# Autodesk Inventor assembly: Final assembly of buggy bot
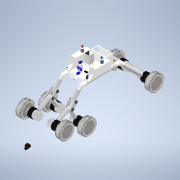
[picture p0: Inventor's stored thumbnail of the model, 180x180]
Saved by Autodesk Inventor 2021 (Build 250183000, 183)
## iProperties
Created: 2021-07-16
Part Number: Final assembly of buggy bot
Document SubType Name: Assembly
Designer: HP
Mass: 47107.8 g
Surface Area: 24762.8 cm^2
Volume: 9232.38 cm^3
Density: 5.10246 g/cm^3
Author: HP
## Documents named in this file (26)
- F:\autodesk inventor\MII\Final assembly of buggy bot.iam
- F:\autodesk inventor\MII\Body.ipt
- F:\autodesk inventor\MII\pvc up.ipt
- F:\autodesk inventor\MII\45elbowfinal.ipt
- F:\autodesk inventor\MII\PVC front 1.ipt
- F:\autodesk inventor\MII\HOLDERPVC.ipt
- F:\autodesk inventor\MII\Dc catcher.ipt
- F:\autodesk inventor\MII\DC.ipt
- F:\autodesk inventor\MII\wheel.ipt
- F:\autodesk inventor\MII\Servo.ipt
- F:\autodesk inventor\MII\smoke.ipt
- F:\autodesk inventor\MII\tilt.ipt
- F:\autodesk inventor\MII\dc to dc.ipt
- F:\autodesk inventor\MII\hbridge.ipt
- F:\autodesk inventor\MII\holder.ipt
- F:\autodesk inventor\MII\bolt.ipt
- F:\autodesk inventor\MII\elbow.ipt
- F:\autodesk inventor\MII\PVC front.ipt
- F:\autodesk inventor\Buggy bot assembly file\Arduino board.ipt
- F:\autodesk inventor\MII\ultrasonic sensor.ipt
- F:\autodesk inventor\MII\temperature sensor.ipt
- F:\autodesk inventor\Water tank.ipt
- F:\autodesk inventor\MII\LED - Copy.ipt
- F:\autodesk inventor\MII\Buzzer.ipt
- F:\autodesk inventor\MII\LED.ipt
- F:\autodesk inventor\Obstacle stone.ipt
## Components (57 placed, 25 different names)
1. Body:1 — Tangent:1, Tangent:2, Flush:1, Flush:2, Angle:2, Tangent:6, Tangent:7, Flush:3, Angle:6, Mate:88, Mate:89, Rigid:8, Angle:7, Angle:10, Angle:11, Insert:1, Rigid:17, Mate:157, Rigid:19, Rotational:2, Rigid:20, Rigid:21, Rigid:22, Rigid:23, Rotational:3
2. pvc up:1 — Tangent:1, Tangent:2, Flush:1, Flush:2, Mate:1, Mate:2, Mate:3, Mate:4
3. 45elbowfinal:1 — Mate:3, Mate:4, Mate:10, Mate:11
4. 45elbowfinal:2 — Mate:1, Mate:2, Mate:13, Mate:14
5. PVC front 1:2 — Mate:10, Mate:11, Mate:43, Rigid:6
6. HOLDERPVC:1 — Mate:13, Mate:14, Mate:92, Mate:93, Tangent:8
7. Dc catcher:2 — Mate:43, Rigid:6, Angle:2, Mate:47, Mate:48
8. DC:5 — Mate:47, Mate:48, Mate:49, Mate:50
9. wheel:1 — Mate:49, Mate:50, Angle:12, Angle:13
10. pvc up:2 — Tangent:6, Tangent:7, Flush:3, Mate:69, Mate:70, Mate:78, Mate:79
11. 45elbowfinal:3 — Mate:69, Mate:70, Mate:71, Mate:72
12. PVC front 1:3 — Mate:71, Mate:72, Mate:73, Rigid:7
13. Dc catcher:9 — Mate:73, Rigid:7, Angle:6, Mate:74, Mate:75
14. DC:8 — Mate:74, Mate:75, Mate:76, Mate:77
15. wheel:6 — Mate:76, Mate:77, Angle:15
16. 45elbowfinal:4 — Mate:78, Mate:79, Mate:80, Mate:81
17. HOLDERPVC:2 — Mate:80, Mate:81, Mate:109, Mate:110, Tangent:11, Tangent:12, Mate:111
18. Servo:1 — Rigid:22
19. smoke:1 — Mate:88, Insert:1
20. tilt:1 — Mate:89
21. dc to dc:1 — Rigid:8
22. hbridge:1 — Mate:157
23. holder:1 — Mate:92, Mate:94, Mate:95, Angle:7, Angle:8, Tangent:8, Mate:97, Mate:100, Tangent:9
24. holder:2 — Mate:93, Mate:96, Angle:8, Mate:98, Tangent:10
25. holder:3 — Mate:110, Tangent:11, Angle:10, Mate:112, Mate:113, Mate:115, Mate:116
26. holder:4 — Mate:109, Tangent:12, Angle:11, Mate:114, Tangent:13
27. bolt:1 — Mate:94, Mate:95, Mate:96
28. elbow:1 — Mate:113, Mate:114, Tangent:13, Mate:128, Mate:129, Mate:131, Mate:132
29. elbow:2 — Mate:97, Mate:98, Mate:99, Tangent:9, Tangent:10, Mate:125, Mate:126, Mate:130, Mate:133
30. bolt:2 — Mate:99, Mate:100
31. bolt:3 — Mate:111, Mate:112
32. bolt:4 — Mate:115, Mate:116
33. PVC front:1 — Mate:125, Mate:126, Mate:127, Mate:146
34. Dc catcher:10 — Mate:127, Mate:146
35. DC:9
36. wheel:7 — Angle:12, Angle:13, Angle:14
37. PVC front:4 — Mate:128, Mate:131, Mate:142, Mate:145
38. PVC front:5 — Mate:130, Mate:133, Mate:140, Mate:141
39. PVC front:6 — Mate:129, Mate:132, Mate:143, Mate:144
40. Dc catcher:11 — Mate:140, Mate:141
41. DC:10 — Mate:147, Mate:148
42. Dc catcher:12 — Mate:143, Mate:144
43. DC:11 — Mate:149, Mate:151
44. Dc catcher:13 — Mate:142, Mate:145
45. DC:12 — Mate:150, Mate:152
46. wheel:8 — Angle:14, Mate:147, Mate:148
47. wheel:9 — Mate:150, Mate:152, Angle:15, Angle:16
48. wheel:10 — Mate:149, Mate:151, Angle:16
49. Arduino board:1 — Rigid:17
50. ultrasonic sensor:1 — Insert:2
51. temperature sensor:1 — Rigid:20
52. Water tank:1 — Rigid:19
53. LED - Copy:1 — Rotational:2
54. Buzzer:1 — Rigid:21
55. Servo:2 — Rigid:23, Insert:2
56. LED:1 — Rotational:3
57. Obstacle stone:1
## Relationships (118: Mate 78, WeldJoint 12, Angle 11, Tangent 10, Flush 3, Insert 2, RevoluteJoint 2)
- Tangent:1: Body:1 ↔ pvc up:1
- Tangent:2: Body:1 ↔ pvc up:1
- Flush:1: Body:1 ↔ pvc up:1
- Flush:2: Body:1 ↔ pvc up:1
- Mate:1: pvc up:1 ↔ 45elbowfinal:2
- Mate:2: pvc up:1 ↔ 45elbowfinal:2
- Mate:3: pvc up:1 ↔ 45elbowfinal:1
- Mate:4: pvc up:1 ↔ 45elbowfinal:1
- Mate:10: 45elbowfinal:1 ↔ PVC front 1:2
- Mate:11: 45elbowfinal:1 ↔ PVC front 1:2
- Mate:13: 45elbowfinal:2 ↔ HOLDERPVC:1
- Mate:14: 45elbowfinal:2 ↔ HOLDERPVC:1
- Mate:43: PVC front 1:2 ↔ Dc catcher:2
- Rigid:6 [WeldJoint]: PVC front 1:2 ↔ Dc catcher:2
- Angle:2 (0 deg): Body:1 ↔ Dc catcher:2
- Mate:47: Dc catcher:2 ↔ DC:5
- Mate:48: Dc catcher:2 ↔ DC:5
- Mate:49: DC:5 ↔ wheel:1
- Mate:50 (5 mm): DC:5 ↔ wheel:1
- Tangent:6: Body:1 ↔ pvc up:2
- Tangent:7: Body:1 ↔ pvc up:2
- Flush:3: Body:1 ↔ pvc up:2
- Mate:69: pvc up:2 ↔ 45elbowfinal:3
- Mate:70: pvc up:2 ↔ 45elbowfinal:3
- Mate:71: 45elbowfinal:3 ↔ PVC front 1:3
- Mate:72: 45elbowfinal:3 ↔ PVC front 1:3
- Mate:73: PVC front 1:3 ↔ Dc catcher:9
- Rigid:7 [WeldJoint]: PVC front 1:3 ↔ Dc catcher:9
- Angle:6 (0 deg): Body:1 ↔ Dc catcher:9
- Mate:74: Dc catcher:9 ↔ DC:8
- Mate:75: Dc catcher:9 ↔ DC:8
- Mate:76: DC:8 ↔ wheel:6
- Mate:77 (5 mm): DC:8 ↔ wheel:6
- Mate:78: pvc up:2 ↔ 45elbowfinal:4
- Mate:79: pvc up:2 ↔ 45elbowfinal:4
- Mate:80: 45elbowfinal:4 ↔ HOLDERPVC:2
- Mate:81: 45elbowfinal:4 ↔ HOLDERPVC:2
- Mate:88: Body:1 ↔ smoke:1
- Mate:89 (5 mm): Body:1 ↔ tilt:1
- Rigid:8 [WeldJoint] (1 mm): Body:1 ↔ dc to dc:1
- Mate:92: HOLDERPVC:1 ↔ holder:1
- Mate:93: HOLDERPVC:1 ↔ holder:2
- Mate:94: holder:1 ↔ bolt:1
- Mate:95 (1 mm): holder:1 ↔ bolt:1
- Mate:96 (10 mm): holder:2 ↔ bolt:1
- Angle:7 (0 deg): Body:1 ↔ holder:1
- Angle:8 (0 deg): holder:1 ↔ holder:2
- Tangent:8 (1 mm): HOLDERPVC:1 ↔ holder:1
- Mate:97: holder:1 ↔ elbow:2
- Mate:98: holder:2 ↔ elbow:2
- Mate:99: elbow:2 ↔ bolt:2
- Mate:100 (1 mm): holder:1 ↔ bolt:2
- Tangent:9: holder:1 ↔ elbow:2
- Tangent:10: holder:2 ↔ elbow:2
- Mate:109: HOLDERPVC:2 ↔ holder:4
- Mate:110: HOLDERPVC:2 ↔ holder:3
- Tangent:11: HOLDERPVC:2 ↔ holder:3
- Tangent:12: HOLDERPVC:2 ↔ holder:4
- Angle:10 (0 deg): Body:1 ↔ holder:3
- Angle:11 (0 deg): Body:1 ↔ holder:4
- Mate:111: HOLDERPVC:2 ↔ bolt:3
- Mate:112 (1 mm): holder:3 ↔ bolt:3
- Mate:113: holder:3 ↔ elbow:1
- Mate:114: holder:4 ↔ elbow:1
- Tangent:13: holder:4 ↔ elbow:1
- Mate:115: holder:3 ↔ bolt:4
- Mate:116 (1 mm): holder:3 ↔ bolt:4
- [Mate]: Dc catcher:10 ↔ DC:9
- [Mate]: Dc catcher:10 ↔ DC:9
- [Mate]: DC:9 ↔ wheel:7
- [Mate] (5 mm): DC:9 ↔ wheel:7
- Angle:12 (0 deg): wheel:1 ↔ wheel:7
- Mate:125: elbow:2 ↔ PVC front:1
- Mate:126: elbow:2 ↔ PVC front:1
- Mate:127: PVC front:1 ↔ Dc catcher:10
- Angle:13 (0 deg): wheel:1 ↔ wheel:7
- Mate:128: elbow:1 ↔ PVC front:4
- Mate:129: elbow:1 ↔ PVC front:6
- Mate:130: elbow:2 ↔ PVC front:5
- Mate:131: elbow:1 ↔ PVC front:4
- Mate:132: elbow:1 ↔ PVC front:6
- Mate:133: elbow:2 ↔ PVC front:5
- [Mate]: Dc catcher:11 ↔ DC:10
- [Mate]: Dc catcher:11 ↔ DC:10
- [WeldJoint]: Dc catcher:11 ↔ DC:10
- [Mate]: Dc catcher:12 ↔ DC:11
- [Mate]: Dc catcher:12 ↔ DC:11
- [WeldJoint]: Dc catcher:12 ↔ DC:11
- [Mate]: Dc catcher:13 ↔ DC:12
- [Mate]: Dc catcher:13 ↔ DC:12
- [WeldJoint]: Dc catcher:13 ↔ DC:12
- Mate:140: PVC front:5 ↔ Dc catcher:11
- Mate:141: PVC front:5 ↔ Dc catcher:11
- Mate:142: PVC front:4 ↔ Dc catcher:13
- Mate:143: PVC front:6 ↔ Dc catcher:12
- Mate:144: PVC front:6 ↔ Dc catcher:12
- Mate:145: PVC front:4 ↔ Dc catcher:13
- Angle:14 (0 deg): wheel:7 ↔ wheel:8
- Mate:146: PVC front:1 ↔ Dc catcher:10
- Mate:147: DC:10 ↔ wheel:8
- Mate:148 (5 mm): DC:10 ↔ wheel:8
- Mate:149: DC:11 ↔ wheel:10
- Mate:150: DC:12 ↔ wheel:9
- Mate:151 (5 mm): DC:11 ↔ wheel:10
- Mate:152 (5 mm): DC:12 ↔ wheel:9
- Angle:15 (0 deg): wheel:6 ↔ wheel:9
- Angle:16 (0 deg): wheel:9 ↔ wheel:10
- Insert:1 (-5 mm): Body:1 ↔ smoke:1
- Rigid:17 [WeldJoint]: Body:1 ↔ Arduino board:1
- Mate:157: Body:1 ↔ hbridge:1
- Rigid:19 [WeldJoint]: Body:1 ↔ Water tank:1
- Rotational:2 [RevoluteJoint] (-1 mm): Body:1 ↔ LED - Copy:1
- Rigid:20 [WeldJoint] (5 mm): Body:1 ↔ temperature sensor:1
- Rigid:21 [WeldJoint]: Body:1 ↔ Buzzer:1
- Rigid:22 [WeldJoint]: Body:1 ↔ Servo:1
- Rigid:23 [WeldJoint]: Body:1 ↔ Servo:2
- Insert:2 (-5 mm): ultrasonic sensor:1 ↔ Servo:2
- Rotational:3 [RevoluteJoint] (-1 mm): Body:1 ↔ LED:1
## Named parameters: d385_d127 = 0 mm, d386_d128 = 0 mm, d387_d129 = 0 mm, d388_d130 = 5 mm, d477_d391 = 0 mm, d478_d385_d127 = 0 mm, d479_d386_d128 = 0 mm, d480_d391 = 0 mm, d481_d385_d127 = 0 mm, d482_d386_d128 = 0 mm, d483_d391 = 0 mm, d484_d385_d127 = 0 mm, d485_d386_d128 = 0 mm
